# Autodesk Inventor assembly: 20mm Gantry Set
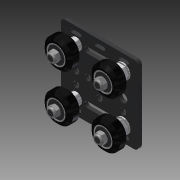
[picture p0: Inventor's stored thumbnail of the model, 180x180]
Saved by Autodesk Inventor 2014 SP1 (Build 180222100, 222)
## iProperties
Created: 2016-04-10
Part Number: 20mm Gantry Set
Document SubType Name: Assembly
Designer: Ben
Author: Ben
## Documents named in this file (6)
- C:\Users\Ben\Documents\Autodesk\Projects\Me\3D printer\carriages\stp\Inventor\20mm Gantry Set.iam
- C:\Users\Ben\Documents\Autodesk\Projects\Me\3D printer\20mm gantry plate.ipt
- C:\Users\Ben\Documents\Autodesk\Projects\Me\3D printer\carriages\V-Wheel Solid Wheel.iam
- C:\Users\Ben\Documents\Autodesk\Projects\Me\3D printer\carriages\V-Wheel Solid Wheel - spacer.iam
- C:\Users\Ben\Documents\Autodesk\Projects\Me\3D printer\carriages\M5x25 low profile screw.ipt
- C:\Users\Ben\Documents\Autodesk\Projects\hardware\Fasteners\M5\M5 Nylock.ipt
## Components (13 placed, 5 different names)
1. 20mm gantry plate:1 — Mate:3, Mate:4, Mate:5, Mate:6, Mate:7, Mate:8, Mate:9, Mate:10, Mate:13, Mate:17, Mate:18, Mate:27, Angle:1, Flush:1, Mate:30, Mate:31, Mate:32, Flush:37, Flush:36
2. V-Wheel Solid Wheel:3 [sub-assembly] — Mate:3, Mate:7, Mate:12, Mate:26
3. V-Wheel Solid Wheel:4 [sub-assembly] — Mate:4, Mate:8, Mate:11, Mate:23
4. V-Wheel Solid Wheel - spacer:1 [sub-assembly] — Mate:5, Mate:10, Mate:25
5. V-Wheel Solid Wheel - spacer:2 [sub-assembly] — Mate:6, Mate:9, Mate:24
6. M5x25 low profile screw:1 — Mate:11, Mate:18, Mate:19
7. M5x25 low profile screw:2 — Mate:12, Mate:17, Mate:20
8. M5x25 low profile screw:3 — Mate:13, Mate:22, Mate:30
9. M5 Nylock:1 — Mate:19, Mate:23
10. M5 Nylock:2 — Mate:20, Mate:26
11. M5 Nylock:3 — Mate:25, Mate:33
12. M5 Nylock:4 — Mate:22, Mate:24
13. M5x25 low profile screw:4 — Mate:31, Mate:32, Mate:33
## Relationships (30: Mate 25, Flush 4, Angle 1)
- Mate:3: 20mm gantry plate:1 ↔ V-Wheel Solid Wheel:3
- Mate:4: 20mm gantry plate:1 ↔ V-Wheel Solid Wheel:4
- Mate:5: 20mm gantry plate:1 ↔ V-Wheel Solid Wheel - spacer:1
- Mate:6: 20mm gantry plate:1 ↔ V-Wheel Solid Wheel - spacer:2
- Mate:7: 20mm gantry plate:1 ↔ V-Wheel Solid Wheel:3
- Mate:8: 20mm gantry plate:1 ↔ V-Wheel Solid Wheel:4
- Mate:9: 20mm gantry plate:1 ↔ V-Wheel Solid Wheel - spacer:2
- Mate:10: 20mm gantry plate:1 ↔ V-Wheel Solid Wheel - spacer:1
- Mate:11: V-Wheel Solid Wheel:4 ↔ M5x25 low profile screw:1
- Mate:12: V-Wheel Solid Wheel:3 ↔ M5x25 low profile screw:2
- Mate:13: 20mm gantry plate:1 ↔ M5x25 low profile screw:3
- Mate:17: 20mm gantry plate:1 ↔ M5x25 low profile screw:2
- Mate:18: 20mm gantry plate:1 ↔ M5x25 low profile screw:1
- Mate:19: M5x25 low profile screw:1 ↔ M5 Nylock:1
- Mate:20: M5x25 low profile screw:2 ↔ M5 Nylock:2
- Mate:22: M5x25 low profile screw:3 ↔ M5 Nylock:4
- Mate:23: V-Wheel Solid Wheel:4 ↔ M5 Nylock:1
- Mate:24: V-Wheel Solid Wheel - spacer:2 ↔ M5 Nylock:4
- Mate:25: V-Wheel Solid Wheel - spacer:1 ↔ M5 Nylock:3
- Mate:26: V-Wheel Solid Wheel:3 ↔ M5 Nylock:2
- Mate:27: 20mm gantry plate:1
- Angle:1 (0 deg): 20mm gantry plate:1
- Flush:1 (11.885 mm): 20mm gantry plate:1
- Mate:30: 20mm gantry plate:1 ↔ M5x25 low profile screw:3
- Mate:31: 20mm gantry plate:1 ↔ M5x25 low profile screw:4
- Mate:32: 20mm gantry plate:1 ↔ M5x25 low profile screw:4
- Mate:33: M5 Nylock:3 ↔ M5x25 low profile screw:4
- Flush:2
- Flush:37: 20mm gantry plate:1
- Flush:36: 20mm gantry plate:1
